# Autodesk Inventor assembly: Картер всборе
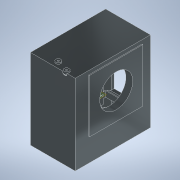
[picture p0: Inventor's stored thumbnail of the model, 180x180]
Saved by Autodesk Inventor 2021 (Build 250183000, 183)
## iProperties
Created: 2020-12-05
Part Number: Картер всборе
Document SubType Name: Assembly
Designer: Тимоха
Author: Тимоха
## Documents named in this file (4)
- C:\Users\Тимоха\Desktop\КР Компрессор\compressor\Картер всборе.iam
- C:\Users\Тимоха\Desktop\КР Компрессор\compressor\Картер.ipt
- C:\Users\Тимоха\Desktop\КР Компрессор\compressor\Крышка коренного подшипника1.ipt
- C:\Users\Тимоха\Desktop\КР Компрессор\compressor\Балка.ipt
## Components (5 placed, 3 different names)
1. Картер:1 — Заподлицо:1, Заподлицо:2, Жесткий:1, Жесткий:2, Жесткий:3
2. Крышка коренного подшипника1:1 — Заподлицо:1, Заподлицо:2
3. Крышка коренного подшипника1:2 — Жесткий:1
4. Балка:1 — Жесткий:2
5. Балка:2 — Жесткий:3
## Relationships (5: WeldJoint 3, Flush 2)
- Заподлицо:1 [Flush]: Картер:1 ↔ Крышка коренного подшипника1:1
- Заподлицо:2 [Flush]: Картер:1 ↔ Крышка коренного подшипника1:1
- Жесткий:1 [WeldJoint]: Картер:1 ↔ Крышка коренного подшипника1:2
- Жесткий:2 [WeldJoint]: Картер:1 ↔ Балка:1
- Жесткий:3 [WeldJoint]: Картер:1 ↔ Балка:2
